# Autodesk Inventor assembly: Drive Roller Assembly 2
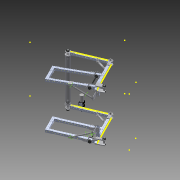
[picture p0: Inventor's stored thumbnail of the model, 180x180]
Saved by Autodesk Inventor 2014 (Build 180170000, 170)
## iProperties
Created: 2014-01-12
Part Number: Drive Roller Assembly 2
Document SubType Name: Assembly
Designer: Michael
Mass: 4835.9 g
Surface Area: 14934.6 cm^2
Volume: 1370.56 cm^3
Density: 3.52842 g/cm^3
Author: Michael
## Documents named in this file (33)
- C:\Users\Michael\Documents\GitHub\2014buildCAD\New Collector\Drive Roller Assembly 2.iam
- C:\Users\Michael\Documents\GitHub\2014buildCAD\Collector\Hex Shaft Collar 1-2 in (7552K500).ipt
- C:\Users\Michael\Documents\GitHub\2014buildCAD\Collector\Roller End Cap Drive (3-D Printed).ipt
- C:\Users\Michael\Documents\GitHub\2014buildCAD\Collector\Vex Pro VersaPlanetary Side Mount.ipt
- C:\Users\Michael\Documents\GitHub\2014buildCAD\Collector\VersaPlanetary (Fixed).iam
- C:\Users\Michael\Documents\GitHub\2014buildCAD\New Collector\Polycarbonate Roller 2 OD 1-16 Thick (8585K64).ipt
- C:\Users\Michael\Documents\GitHub\2014buildCAD\New Collector\Hex Bearing 1-2 in (FR8ZZ-Hex, am-0279).ipt
- C:\Users\Michael\Documents\GitHub\2014buildCAD\New Collector\Hex Shaft Collar 1-2 in (7552K500).ipt
- C:\Users\Michael\Documents\GitHub\2014buildCAD\New Collector\Roller End Cap Drive (3-D Printed).ipt
- C:\Users\Michael\Documents\GitHub\2014buildCAD\New Collector\Vex Pro End Bearing Mount.ipt
- C:\Users\Michael\Documents\GitHub\2014buildCAD\New Collector\Vex Pro 1x1 rectangular tubing 14 in length.ipt
- C:\Users\Michael\Documents\GitHub\2014buildCAD\New Collector\Hex Shaft Aluminum 1-2 in (am-2291).ipt
- C:\Users\Michael\Documents\GitHub\2014buildCAD\New Collector\Timing Pulley (HTD 5mm) - 18T 9mm Double Flange, 1-2 in Hex (VexPro).ipt
- C:\Users\Michael\Documents\GitHub\2014buildCAD\New Collector\Clamp with Piston Assembly.iam
- C:\Users\Michael\Documents\GitHub\2014buildCAD\New Collector\Vex Pro 90 degree gusset.ipt
- C:\Users\Michael\Documents\GitHub\2014buildCAD\New Collector\Vex Pro 1x1 rectangular tubing 2 in length.ipt
- C:\Users\Michael\Documents\GitHub\2014buildCAD\New Collector\Hex Shaft 3-8 in (am-0855).ipt
- C:\Users\Michael\Documents\GitHub\2014buildCAD\New Collector\Hex Shaft Collar 3-8 in (7552K300).ipt
- C:\Users\Michael\Documents\GitHub\2014buildCAD\New Collector\3 Postion Pneumatic Cylinder (9-16 in Bore, .25 in,2 in stroke).iam
- C:\Users\Michael\Documents\GitHub\2014buildCAD\New Collector\Hex Shaft 1-2 in (am-0856).ipt
- C:\Users\Michael\Documents\GitHub\2014buildCAD\New Collector\Spacer 2.ipt
- C:\Users\Michael\Documents\GitHub\2014buildCAD\New Collector\Gusset 3 (R-R) (Custom) ipt.ipt
- C:\Users\Michael\Documents\GitHub\2014buildCAD\New Collector\Gusset 3 (L-R) (Custom).ipt
- C:\Users\Michael\Documents\GitHub\2014buildCAD\New Collector\Gusset 3 (L-L) (Custom) ipt.ipt
- C:\Users\Michael\Documents\GitHub\2014buildCAD\New Collector\Gusset 3 (R-L) (Custom).ipt
- C:\Users\Michael\Documents\GitHub\2014buildCAD\New Collector\Vex Pro 1x1 rectangular tubing 4 in length.ipt
- C:\Users\Michael\Documents\GitHub\2014buildCAD\New Collector\Pneumatic Piston Back Flange (Lt Custom).ipt
- C:\Users\Michael\Documents\GitHub\2014buildCAD\New Collector\Pneumatic Piston Front Flange (Lt Custom).ipt
- C:\Users\Michael\Documents\GitHub\2014buildCAD\New Collector\Pneumatic Piston Front Flange (Rt Custom).ipt
- C:\Users\Michael\Documents\GitHub\2014buildCAD\New Collector\Pneumatic Piston Back Flange (Rt Custom).ipt
- C:\Users\Michael\Documents\GitHub\2014buildCAD\New Collector\Bearing Mount Spacer 1-8 in.ipt
- C:\Users\Michael\Documents\GitHub\2014buildCAD\New Collector\Vex Pro 1x1 rectangular tubing 14 in length (roller).ipt
- C:\Users\Michael\Documents\GitHub\2014buildCAD\New Collector\Complete Roller Pneumatic Cylinder Assembly.iam
## Components (95 placed, 30 different names)
1. Roller End Cap Drive (3-D Printed):2 — Mate:154, Mate:155, Mate:157, Mate:158, Mate:466, Mate:469
2. Vex Pro VersaPlanetary Side Mount:1 — Insert:29, Insert:30, Mate:564, Mate:565, Mate:566
3. VersaPlanetary (Fixed):1 [sub-assembly] — Insert:29, Insert:30, Mate:113, Mate:114, Mate:120, Mate:121, Mate:153
4. Hex Shaft Collar 1-2 in (7552K500):9 — Mate:113, Mate:114
5. Hex Shaft Collar 1-2 in (7552K500):10 — Mate:120, Mate:121
6. Polycarbonate Roller 2 OD 1-16 Thick (8585K64):3 — Mate:157, Mate:158, Mate:159, Mate:160
7. Hex Bearing 1-2 in (FR8ZZ-Hex, am-0279):3 — Mate:128, Mate:129, Mate:134, Mate:466
8. Roller End Cap Drive (3-D Printed):5 — Mate:159, Mate:160, Mate:632, Mate:635
9. Hex Shaft Aluminum 1-2 in (am-2291):1 — Flush:1, Mate:132, Mate:133, Mate:134, Mate:143, Mate:144, Mate:146, Mate:147, Mate:154, Mate:155, Mate:172, Mate:173, Mate:179, Mate:180, Mate:467, Mate:468
10. Vex Pro End Bearing Mount:4 — Mate:130, Mate:131, Mate:619, Mate:620, Mate:621
11. Vex Pro End Bearing Mount:5 — Mate:128, Mate:129, Mate:622, Mate:623, Mate:624
12. Hex Bearing 1-2 in (FR8ZZ-Hex, am-0279):4 — Mate:130, Mate:131, Flush:1, Mate:132, Mate:133, Mate:161
13. Timing Pulley (HTD 5mm) - 18T 9mm Double Flange, 1-2 in Hex (VexPro):3 — Mate:143, Mate:144, Mate:145, Mate:161
14. Hex Shaft Collar 1-2 in (7552K500):13 — Mate:145, Mate:146, Mate:147, Flush:2
15. Hex Shaft Collar 1-2 in (7552K500):14 — Flush:4, Mate:152
16. Timing Pulley (HTD 5mm) - 18T 9mm Double Flange, 1-2 in Hex (VexPro):4 — Mate:150, Flush:3, Mate:151, Flush:4, Mate:152
17. Hex Shaft Collar 1-2 in (7552K500):15 — Flush:2, Mate:150, Flush:3, Mate:151, Mate:153
18. Hex Bearing 1-2 in (FR8ZZ-Hex, am-0279):5 — Mate:178
19. Vex Pro End Bearing Mount:7 — Mate:626, Mate:630, Mate:631
20. Vex Pro End Bearing Mount:8 — Mate:627, Mate:628, Mate:629
21. Hex Bearing 1-2 in (FR8ZZ-Hex, am-0279):6 — Mate:172, Mate:173, Mate:470, Mate:471, Mate:632
22. Hex Shaft Collar 1-2 in (7552K500):16 — Mate:178, Mate:179, Mate:180, Flush:13
23. Clamp with Piston Assembly:1 [sub-assembly] — Mate:226, Mate:227, Flush:6, Mate:230, Mate:233, Mate:521, Mate:522, Mate:523
24. Vex Pro 1x1 rectangular tubing 14 in length:5 — Mate:203, Mate:210, Mate:211, Mate:221, Mate:222, Mate:223, Mate:264, Mate:265, Mate:266, Mate:267, Mate:268, Mate:269, Mate:326, Mate:328, Mate:329, Mate:427, Mate:429, Mate:611, Mate:612, Mate:615, Mate:616, Mate:617, Mate:618, Flush:20, Mate:644, Mate:648, Mate:649
25. Vex Pro 1x1 rectangular tubing 14 in length:6 — Mate:258, Mate:259, Mate:260, Mate:263, Mate:298, Mate:299, Mate:300, Mate:301, Mate:305, Mate:306, Mate:320, Mate:321, Mate:322, Mate:323, Mate:418, Mate:419, Mate:420, Mate:502, Mate:544, Mate:545, Mate:546, Mate:553, Mate:554, Mate:555, Flush:20, Mate:637, Mate:638, Mate:639, Mate:642
26. Vex Pro 90 degree gusset:8 — Mate:203, Mate:210, Mate:211, Mate:212, Mate:213, Mate:214
27. Vex Pro 1x1 rectangular tubing 2 in length:1 — Mate:212, Mate:213, Mate:214, Mate:327
28. Vex Pro 90 degree gusset:10 — Mate:221, Mate:222, Mate:223, Mate:433, Mate:434, Mate:435
29. Vex Pro 1x1 rectangular tubing 2 in length:2 — Mate:224, Mate:225, Flush:5, Mate:428
30. Hex Shaft 3-8 in (am-0855):1 — Mate:224, Mate:225, Flush:5, Mate:226, Mate:227, Flush:6, Mate:228, Mate:229, Mate:231, Mate:232
31. Hex Shaft Collar 3-8 in (7552K300):1 — Mate:228, Mate:229, Mate:230
32. Hex Shaft Collar 3-8 in (7552K300):2 — Mate:231, Mate:232, Mate:233
33. Clamp with Piston Assembly:2 [sub-assembly] — Mate:509, Mate:510, Mate:511
34. Vex Pro 90 degree gusset:11 — Mate:322, Mate:323, Mate:642
35. Vex Pro 90 degree gusset:12 — Mate:263, Mate:320, Mate:321, Mate:324, Mate:325
36. Vex Pro 1x1 rectangular tubing 2 in length:3 — Mate:324, Mate:325
37. Vex Pro 90 degree gusset:13 — Mate:258, Mate:259, Mate:260, Mate:425, Mate:426, Mate:492
38. Vex Pro 1x1 rectangular tubing 2 in length:4
39. Hex Shaft 3-8 in (am-0855):2
40. Hex Shaft Collar 3-8 in (7552K300):3
41. Hex Shaft Collar 3-8 in (7552K300):4
42. 3 Postion Pneumatic Cylinder (9-16 in Bore, .25 in,2 in stroke):1 [sub-assembly] — Mate:516, Mate:517, Mate:518, Mate:636
43. Vex Pro 90 degree gusset:14 — Mate:264, Mate:265, Mate:266, Mate:476, Mate:477, Mate:478
44. Vex Pro 90 degree gusset:15 — Mate:267, Mate:268, Mate:269
45. Vex Pro 90 degree gusset:17 — Mate:300, Mate:301, Mate:305, Mate:306, Mate:485, Mate:486, Mate:487
46. Vex Pro 90 degree gusset:18 — Mate:298, Mate:299, Mate:502
47. Vex Pro 90 degree gusset:19 — Mate:326, Mate:327, Mate:328, Mate:329
48. Hex Shaft 1-2 in (am-0856):2 — Mate:402, Mate:403, Mate:405, Mate:406, Mate:447, Mate:448, Flush:12
49. Hex Shaft Collar 1-2 in (7552K500):18 — Mate:402, Mate:403, Mate:450, Flush:12
50. Hex Shaft Collar 1-2 in (7552K500):19 — Mate:405, Mate:406, Mate:449
51. Hex Shaft 1-2 in (am-0856):3 — Mate:411, Mate:412, Flush:11, Mate:493, Mate:494, Mate:496, Mate:497
52. Hex Shaft Collar 1-2 in (7552K500):20 — Mate:411, Mate:412, Flush:11, Mate:495
53. Hex Shaft Collar 1-2 in (7552K500):21 — Mate:446, Mate:496, Mate:497
54. Spacer 2:1 — Mate:418, Mate:419, Mate:420, Mate:438, Mate:439, Mate:451, Mate:452, Mate:453
55. Gusset 3 (R-R) (Custom) ipt:1 — Mate:425, Mate:426, Mate:446, Mate:492
56. Spacer 2:2 — Mate:427, Mate:428, Mate:429, Mate:430, Mate:431, Mate:455, Mate:456, Mate:457
57. Gusset 3 (L-R) (Custom):1 — Mate:430, Mate:431, Mate:447, Mate:448, Mate:450, Mate:461
58. Gusset 3 (L-L) (Custom) ipt:1 — Mate:433, Mate:434, Mate:435, Mate:449
59. Gusset 3 (R-L) (Custom):1 — Mate:438, Mate:439, Mate:465, Mate:493, Mate:494, Mate:495
60. Spacer 2:3 — Mate:451, Mate:452, Mate:453, Mate:462, Mate:463, Mate:464
61. Spacer 2:4 — Mate:455, Mate:456, Mate:457, Mate:458, Mate:459, Mate:460
62. Spacer 2:5 — Mate:458, Mate:459, Mate:460, Mate:461
63. Spacer 2:6 — Mate:462, Mate:463, Mate:464, Mate:465
64. Hex Shaft Collar 1-2 in (7552K500):22 — Mate:467, Mate:468, Mate:469
65. Hex Shaft Aluminum 1-2 in (am-2291):2 — Mate:470, Mate:471, Flush:13, Mate:633, Mate:634
66. Vex Pro 1x1 rectangular tubing 4 in length:1 — Mate:476, Mate:477, Mate:478, Mate:513, Mate:514, Mate:515
67. Vex Pro 1x1 rectangular tubing 4 in length:2 — Mate:485, Mate:486, Mate:487, Mate:503, Mate:504, Mate:505
68. 3 Postion Pneumatic Cylinder (9-16 in Bore, .25 in,2 in stroke):2 [sub-assembly] — Mate:506, Mate:507, Mate:508, Mate:512
69. Pneumatic Piston Back Flange (Lt Custom):1 — Mate:503, Mate:504, Mate:505, Mate:506, Mate:507, Mate:508
70. Pneumatic Piston Front Flange (Lt Custom):1 — Mate:509, Mate:510, Mate:511, Mate:512
71. Pneumatic Piston Front Flange (Rt Custom):1 — Mate:521, Mate:522, Mate:523, Mate:636
72. Pneumatic Piston Back Flange (Rt Custom):1 — Mate:513, Mate:514, Mate:515, Mate:516, Mate:517, Mate:518
73. Vex Pro End Bearing Mount:9 — Mate:556, Mate:557
74. Bearing Mount Spacer 1-8 in:1
75. Bearing Mount Spacer 1-8 in:2 — Mate:544, Mate:545, Mate:546
76. Vex Pro End Bearing Mount:10 — Mate:558, Mate:559
77. Bearing Mount Spacer 1-8 in:3
78. Bearing Mount Spacer 1-8 in:4 — Mate:553, Mate:554, Mate:555
79. Hex Bearing 1-2 in (FR8ZZ-Hex, am-0279):7 — Mate:556, Mate:557, Flush:15, Mate:560, Mate:561, Mate:567
80. Hex Shaft 1-2 in (am-0856):4 — Mate:560, Mate:561, Mate:562, Mate:563
81. Hex Bearing 1-2 in (FR8ZZ-Hex, am-0279):8 — Mate:558, Mate:559, Flush:15
82. Vex Pro 1x1 rectangular tubing 14 in length (roller):1 — Mate:562, Mate:563, Mate:564, Mate:565, Mate:566, Mate:567, Mate:619, Mate:620, Mate:621, Mate:622, Mate:623, Mate:624, Flush:21, Mate:640, Mate:641
83. Vex Pro End Bearing Mount:11 — Mate:611, Mate:612
84. Bearing Mount Spacer 1-8 in:5
85. Bearing Mount Spacer 1-8 in:6 — Mate:618
86. Vex Pro End Bearing Mount:12
87. Bearing Mount Spacer 1-8 in:7
88. Bearing Mount Spacer 1-8 in:8 — Mate:615, Mate:616, Mate:617
89. Hex Bearing 1-2 in (FR8ZZ-Hex, am-0279):9 — Flush:19
90. Hex Shaft 1-2 in (am-0856):5 — Flush:19
91. Hex Bearing 1-2 in (FR8ZZ-Hex, am-0279):10
92. Vex Pro 1x1 rectangular tubing 14 in length (roller):2 — Mate:626, Mate:627, Mate:628, Mate:629, Mate:630, Mate:631, Flush:21, Mate:646, Mate:647
93. Hex Shaft Collar 1-2 in (7552K500):23 — Mate:633, Mate:634, Mate:635
94. Complete Roller Pneumatic Cylinder Assembly:1 [sub-assembly] — Mate:637, Mate:638, Mate:639, Mate:640, Mate:641
95. Complete Roller Pneumatic Cylinder Assembly:2 [sub-assembly] — Mate:644, Mate:646, Mate:647, Mate:648, Mate:649
## Relationships (281: Mate 263, Flush 16, Insert 2)
- Insert:29: Vex Pro VersaPlanetary Side Mount:1 ↔ VersaPlanetary (Fixed):1
- Insert:30: Vex Pro VersaPlanetary Side Mount:1 ↔ VersaPlanetary (Fixed):1
- Mate:113: VersaPlanetary (Fixed):1 ↔ Hex Shaft Collar 1-2 in (7552K500):9
- Mate:114: VersaPlanetary (Fixed):1 ↔ Hex Shaft Collar 1-2 in (7552K500):9
- Mate:120: VersaPlanetary (Fixed):1 ↔ Hex Shaft Collar 1-2 in (7552K500):10
- Mate:121: VersaPlanetary (Fixed):1 ↔ Hex Shaft Collar 1-2 in (7552K500):10
- Mate:128: Hex Bearing 1-2 in (FR8ZZ-Hex, am-0279):3 ↔ Vex Pro End Bearing Mount:5
- Mate:129: Hex Bearing 1-2 in (FR8ZZ-Hex, am-0279):3 ↔ Vex Pro End Bearing Mount:5
- Mate:130: Vex Pro End Bearing Mount:4 ↔ Hex Bearing 1-2 in (FR8ZZ-Hex, am-0279):4
- Mate:131: Vex Pro End Bearing Mount:4 ↔ Hex Bearing 1-2 in (FR8ZZ-Hex, am-0279):4
- Flush:1 (-25.4 mm): Hex Shaft Aluminum 1-2 in (am-2291):1 ↔ Hex Bearing 1-2 in (FR8ZZ-Hex, am-0279):4
- Mate:132: Hex Shaft Aluminum 1-2 in (am-2291):1 ↔ Hex Bearing 1-2 in (FR8ZZ-Hex, am-0279):4
- Mate:133: Hex Shaft Aluminum 1-2 in (am-2291):1 ↔ Hex Bearing 1-2 in (FR8ZZ-Hex, am-0279):4
- Mate:134: Hex Bearing 1-2 in (FR8ZZ-Hex, am-0279):3 ↔ Hex Shaft Aluminum 1-2 in (am-2291):1
- Mate:143: Hex Shaft Aluminum 1-2 in (am-2291):1 ↔ Timing Pulley (HTD 5mm) - 18T 9mm Double Flange, 1-2 in Hex (VexPro):3
- Mate:144: Hex Shaft Aluminum 1-2 in (am-2291):1 ↔ Timing Pulley (HTD 5mm) - 18T 9mm Double Flange, 1-2 in Hex (VexPro):3
- Mate:145: Timing Pulley (HTD 5mm) - 18T 9mm Double Flange, 1-2 in Hex (VexPro):3 ↔ Hex Shaft Collar 1-2 in (7552K500):13
- Mate:146: Hex Shaft Aluminum 1-2 in (am-2291):1 ↔ Hex Shaft Collar 1-2 in (7552K500):13
- Mate:147: Hex Shaft Aluminum 1-2 in (am-2291):1 ↔ Hex Shaft Collar 1-2 in (7552K500):13
- [Mate]: Hex Shaft Collar 1-2 in (7552K500):14 ↔ Timing Pulley (HTD 5mm) - 18T 9mm Double Flange, 1-2 in Hex (VexPro):4
- [Mate]: Timing Pulley (HTD 5mm) - 18T 9mm Double Flange, 1-2 in Hex (VexPro):4 ↔ Hex Shaft Collar 1-2 in (7552K500):15
- Flush:2: Hex Shaft Collar 1-2 in (7552K500):13 ↔ Hex Shaft Collar 1-2 in (7552K500):15
- Mate:150: Timing Pulley (HTD 5mm) - 18T 9mm Double Flange, 1-2 in Hex (VexPro):4 ↔ Hex Shaft Collar 1-2 in (7552K500):15
- Flush:3: Timing Pulley (HTD 5mm) - 18T 9mm Double Flange, 1-2 in Hex (VexPro):4 ↔ Hex Shaft Collar 1-2 in (7552K500):15
- Mate:151: Timing Pulley (HTD 5mm) - 18T 9mm Double Flange, 1-2 in Hex (VexPro):4 ↔ Hex Shaft Collar 1-2 in (7552K500):15
- Flush:4: Hex Shaft Collar 1-2 in (7552K500):14 ↔ Timing Pulley (HTD 5mm) - 18T 9mm Double Flange, 1-2 in Hex (VexPro):4
- Mate:152: Hex Shaft Collar 1-2 in (7552K500):14 ↔ Timing Pulley (HTD 5mm) - 18T 9mm Double Flange, 1-2 in Hex (VexPro):4
- Mate:153: VersaPlanetary (Fixed):1 ↔ Hex Shaft Collar 1-2 in (7552K500):15
- Mate:154: Roller End Cap Drive (3-D Printed):2 ↔ Hex Shaft Aluminum 1-2 in (am-2291):1
- Mate:155: Roller End Cap Drive (3-D Printed):2 ↔ Hex Shaft Aluminum 1-2 in (am-2291):1
- Mate:157: Roller End Cap Drive (3-D Printed):2 ↔ Polycarbonate Roller 2 OD 1-16 Thick (8585K64):3
- Mate:158: Roller End Cap Drive (3-D Printed):2 ↔ Polycarbonate Roller 2 OD 1-16 Thick (8585K64):3
- Mate:159: Polycarbonate Roller 2 OD 1-16 Thick (8585K64):3 ↔ Roller End Cap Drive (3-D Printed):5
- Mate:160: Polycarbonate Roller 2 OD 1-16 Thick (8585K64):3 ↔ Roller End Cap Drive (3-D Printed):5
- Mate:161: Hex Bearing 1-2 in (FR8ZZ-Hex, am-0279):4 ↔ Timing Pulley (HTD 5mm) - 18T 9mm Double Flange, 1-2 in Hex (VexPro):3
- [Mate]: Hex Bearing 1-2 in (FR8ZZ-Hex, am-0279):5 ↔ Vex Pro End Bearing Mount:8
- [Mate]: Hex Bearing 1-2 in (FR8ZZ-Hex, am-0279):5 ↔ Vex Pro End Bearing Mount:8
- [Mate]: Vex Pro End Bearing Mount:7 ↔ Hex Bearing 1-2 in (FR8ZZ-Hex, am-0279):6
- [Mate]: Vex Pro End Bearing Mount:7 ↔ Hex Bearing 1-2 in (FR8ZZ-Hex, am-0279):6
- Mate:172: Hex Shaft Aluminum 1-2 in (am-2291):1 ↔ Hex Bearing 1-2 in (FR8ZZ-Hex, am-0279):6
- Mate:173: Hex Shaft Aluminum 1-2 in (am-2291):1 ↔ Hex Bearing 1-2 in (FR8ZZ-Hex, am-0279):6
- Mate:178: Hex Bearing 1-2 in (FR8ZZ-Hex, am-0279):5 ↔ Hex Shaft Collar 1-2 in (7552K500):16
- Mate:179: Hex Shaft Aluminum 1-2 in (am-2291):1 ↔ Hex Shaft Collar 1-2 in (7552K500):16
- Mate:180: Hex Shaft Aluminum 1-2 in (am-2291):1 ↔ Hex Shaft Collar 1-2 in (7552K500):16
- Mate:203: Vex Pro 1x1 rectangular tubing 14 in length:5 ↔ Vex Pro 90 degree gusset:8
- Mate:210: Vex Pro 1x1 rectangular tubing 14 in length:5 ↔ Vex Pro 90 degree gusset:8
- Mate:211: Vex Pro 1x1 rectangular tubing 14 in length:5 ↔ Vex Pro 90 degree gusset:8
- Mate:212: Vex Pro 90 degree gusset:8 ↔ Vex Pro 1x1 rectangular tubing 2 in length:1
- Mate:213: Vex Pro 90 degree gusset:8 ↔ Vex Pro 1x1 rectangular tubing 2 in length:1
- Mate:214: Vex Pro 90 degree gusset:8 ↔ Vex Pro 1x1 rectangular tubing 2 in length:1
- [Mate]: Vex Pro 90 degree gusset:10 ↔ Vex Pro 1x1 rectangular tubing 2 in length:2
- [Mate]: Vex Pro 90 degree gusset:10 ↔ Vex Pro 1x1 rectangular tubing 2 in length:2
- [Mate]: Vex Pro 90 degree gusset:10 ↔ Vex Pro 1x1 rectangular tubing 2 in length:2
- Mate:221: Vex Pro 1x1 rectangular tubing 14 in length:5 ↔ Vex Pro 90 degree gusset:10
- Mate:222: Vex Pro 1x1 rectangular tubing 14 in length:5 ↔ Vex Pro 90 degree gusset:10
- Mate:223: Vex Pro 1x1 rectangular tubing 14 in length:5 ↔ Vex Pro 90 degree gusset:10
- Mate:224: Vex Pro 1x1 rectangular tubing 2 in length:2 ↔ Hex Shaft 3-8 in (am-0855):1
- Mate:225: Vex Pro 1x1 rectangular tubing 2 in length:2 ↔ Hex Shaft 3-8 in (am-0855):1
- Flush:5 (-19.05 mm): Vex Pro 1x1 rectangular tubing 2 in length:2 ↔ Hex Shaft 3-8 in (am-0855):1
- Mate:226: Clamp with Piston Assembly:1 ↔ Hex Shaft 3-8 in (am-0855):1
- Mate:227: Clamp with Piston Assembly:1 ↔ Hex Shaft 3-8 in (am-0855):1
- Flush:6 (-9.525 mm): Clamp with Piston Assembly:1 ↔ Hex Shaft 3-8 in (am-0855):1
- Mate:228: Hex Shaft 3-8 in (am-0855):1 ↔ Hex Shaft Collar 3-8 in (7552K300):1
- Mate:229: Hex Shaft 3-8 in (am-0855):1 ↔ Hex Shaft Collar 3-8 in (7552K300):1
- Mate:230: Clamp with Piston Assembly:1 ↔ Hex Shaft Collar 3-8 in (7552K300):1
- Mate:231: Hex Shaft 3-8 in (am-0855):1 ↔ Hex Shaft Collar 3-8 in (7552K300):2
- Mate:232: Hex Shaft 3-8 in (am-0855):1 ↔ Hex Shaft Collar 3-8 in (7552K300):2
- Mate:233: Clamp with Piston Assembly:1 ↔ Hex Shaft Collar 3-8 in (7552K300):2
- [Mate]: Vex Pro 90 degree gusset:12 ↔ Vex Pro 1x1 rectangular tubing 2 in length:3
- [Mate]: Vex Pro 90 degree gusset:13 ↔ Vex Pro 1x1 rectangular tubing 2 in length:4
- [Mate]: Vex Pro 90 degree gusset:13 ↔ Vex Pro 1x1 rectangular tubing 2 in length:4
- [Mate]: Vex Pro 90 degree gusset:13 ↔ Vex Pro 1x1 rectangular tubing 2 in length:4
- [Mate]: Vex Pro 1x1 rectangular tubing 2 in length:4 ↔ Hex Shaft 3-8 in (am-0855):2
- [Mate]: Vex Pro 1x1 rectangular tubing 2 in length:4 ↔ Hex Shaft 3-8 in (am-0855):2
- [Flush] (-19.05 mm): Vex Pro 1x1 rectangular tubing 2 in length:4 ↔ Hex Shaft 3-8 in (am-0855):2
- [Mate]: Clamp with Piston Assembly:2 ↔ Hex Shaft 3-8 in (am-0855):2
- [Mate]: Clamp with Piston Assembly:2 ↔ Hex Shaft 3-8 in (am-0855):2
- [Flush] (-9.525 mm): Clamp with Piston Assembly:2 ↔ Hex Shaft 3-8 in (am-0855):2
- [Mate]: Hex Shaft 3-8 in (am-0855):2 ↔ Hex Shaft Collar 3-8 in (7552K300):3
- [Mate]: Hex Shaft 3-8 in (am-0855):2 ↔ Hex Shaft Collar 3-8 in (7552K300):3
- [Mate]: Clamp with Piston Assembly:2 ↔ Hex Shaft Collar 3-8 in (7552K300):3
- [Mate]: Hex Shaft 3-8 in (am-0855):2 ↔ Hex Shaft Collar 3-8 in (7552K300):4
- [Mate]: Hex Shaft 3-8 in (am-0855):2 ↔ Hex Shaft Collar 3-8 in (7552K300):4
- [Mate]: Clamp with Piston Assembly:2 ↔ Hex Shaft Collar 3-8 in (7552K300):4
- Mate:258: Vex Pro 1x1 rectangular tubing 14 in length:6 ↔ Vex Pro 90 degree gusset:13
- Mate:259: Vex Pro 1x1 rectangular tubing 14 in length:6 ↔ Vex Pro 90 degree gusset:13
- Mate:260: Vex Pro 1x1 rectangular tubing 14 in length:6 ↔ Vex Pro 90 degree gusset:13
- Mate:263: Vex Pro 1x1 rectangular tubing 14 in length:6 ↔ Vex Pro 90 degree gusset:12
- Mate:264: Vex Pro 1x1 rectangular tubing 14 in length:5 ↔ Vex Pro 90 degree gusset:14
- Mate:265: Vex Pro 1x1 rectangular tubing 14 in length:5 ↔ Vex Pro 90 degree gusset:14
- Mate:266: Vex Pro 1x1 rectangular tubing 14 in length:5 ↔ Vex Pro 90 degree gusset:14
- Mate:267: Vex Pro 1x1 rectangular tubing 14 in length:5 ↔ Vex Pro 90 degree gusset:15
- Mate:268: Vex Pro 1x1 rectangular tubing 14 in length:5 ↔ Vex Pro 90 degree gusset:15
- Mate:269: Vex Pro 1x1 rectangular tubing 14 in length:5 ↔ Vex Pro 90 degree gusset:15
- Mate:298: Vex Pro 1x1 rectangular tubing 14 in length:6 ↔ Vex Pro 90 degree gusset:18
- Mate:299: Vex Pro 1x1 rectangular tubing 14 in length:6 ↔ Vex Pro 90 degree gusset:18
- Mate:300: Vex Pro 1x1 rectangular tubing 14 in length:6 ↔ Vex Pro 90 degree gusset:17
- Mate:301: Vex Pro 1x1 rectangular tubing 14 in length:6 ↔ Vex Pro 90 degree gusset:17
- Mate:305: Vex Pro 1x1 rectangular tubing 14 in length:6 ↔ Vex Pro 90 degree gusset:17
- Mate:306: Vex Pro 1x1 rectangular tubing 14 in length:6 ↔ Vex Pro 90 degree gusset:17
- Mate:320: Vex Pro 1x1 rectangular tubing 14 in length:6 ↔ Vex Pro 90 degree gusset:12
- Mate:321: Vex Pro 1x1 rectangular tubing 14 in length:6 ↔ Vex Pro 90 degree gusset:12
- Mate:322: Vex Pro 1x1 rectangular tubing 14 in length:6 ↔ Vex Pro 90 degree gusset:11
- Mate:323: Vex Pro 1x1 rectangular tubing 14 in length:6 ↔ Vex Pro 90 degree gusset:11
- Mate:324: Vex Pro 90 degree gusset:12 ↔ Vex Pro 1x1 rectangular tubing 2 in length:3
- Mate:325: Vex Pro 90 degree gusset:12 ↔ Vex Pro 1x1 rectangular tubing 2 in length:3
- Mate:326: Vex Pro 1x1 rectangular tubing 14 in length:5 ↔ Vex Pro 90 degree gusset:19
- Mate:327: Vex Pro 1x1 rectangular tubing 2 in length:1 ↔ Vex Pro 90 degree gusset:19
- Mate:328: Vex Pro 1x1 rectangular tubing 14 in length:5 ↔ Vex Pro 90 degree gusset:19
- Mate:329: Vex Pro 1x1 rectangular tubing 14 in length:5 ↔ Vex Pro 90 degree gusset:19
- Mate:402: Hex Shaft 1-2 in (am-0856):2 ↔ Hex Shaft Collar 1-2 in (7552K500):18
- Mate:403: Hex Shaft 1-2 in (am-0856):2 ↔ Hex Shaft Collar 1-2 in (7552K500):18
- Mate:405: Hex Shaft 1-2 in (am-0856):2 ↔ Hex Shaft Collar 1-2 in (7552K500):19
- Mate:406: Hex Shaft 1-2 in (am-0856):2 ↔ Hex Shaft Collar 1-2 in (7552K500):19
- Mate:411: Hex Shaft 1-2 in (am-0856):3 ↔ Hex Shaft Collar 1-2 in (7552K500):20
- Mate:412: Hex Shaft 1-2 in (am-0856):3 ↔ Hex Shaft Collar 1-2 in (7552K500):20
- Flush:11 (-9.525 mm): Hex Shaft 1-2 in (am-0856):3 ↔ Hex Shaft Collar 1-2 in (7552K500):20
- Mate:418: Vex Pro 1x1 rectangular tubing 14 in length:6 ↔ Spacer 2:1
- Mate:419: Vex Pro 1x1 rectangular tubing 14 in length:6 ↔ Spacer 2:1
- Mate:420: Vex Pro 1x1 rectangular tubing 14 in length:6 ↔ Spacer 2:1
- Mate:425: Vex Pro 90 degree gusset:13 ↔ Gusset 3 (R-R) (Custom) ipt:1
- Mate:426: Vex Pro 90 degree gusset:13 ↔ Gusset 3 (R-R) (Custom) ipt:1
- Mate:427: Vex Pro 1x1 rectangular tubing 14 in length:5 ↔ Spacer 2:2
- Mate:428: Vex Pro 1x1 rectangular tubing 2 in length:2 ↔ Spacer 2:2
- Mate:429: Vex Pro 1x1 rectangular tubing 14 in length:5 ↔ Spacer 2:2
- Mate:430: Spacer 2:2 ↔ Gusset 3 (L-R) (Custom):1
- Mate:431: Spacer 2:2 ↔ Gusset 3 (L-R) (Custom):1
- Mate:433: Vex Pro 90 degree gusset:10 ↔ Gusset 3 (L-L) (Custom) ipt:1
- Mate:434: Vex Pro 90 degree gusset:10 ↔ Gusset 3 (L-L) (Custom) ipt:1
- Mate:435: Vex Pro 90 degree gusset:10 ↔ Gusset 3 (L-L) (Custom) ipt:1
- Mate:438: Spacer 2:1 ↔ Gusset 3 (R-L) (Custom):1
- Mate:439: Spacer 2:1 ↔ Gusset 3 (R-L) (Custom):1
- Mate:446: Hex Shaft Collar 1-2 in (7552K500):21 ↔ Gusset 3 (R-R) (Custom) ipt:1
- Mate:447: Hex Shaft 1-2 in (am-0856):2 ↔ Gusset 3 (L-R) (Custom):1
- Mate:448: Hex Shaft 1-2 in (am-0856):2 ↔ Gusset 3 (L-R) (Custom):1
- Mate:449: Hex Shaft Collar 1-2 in (7552K500):19 ↔ Gusset 3 (L-L) (Custom) ipt:1
- Mate:450: Hex Shaft Collar 1-2 in (7552K500):18 ↔ Gusset 3 (L-R) (Custom):1
- Mate:451: Spacer 2:1 ↔ Spacer 2:3
- Mate:452: Spacer 2:1 ↔ Spacer 2:3
- Mate:453: Spacer 2:1 ↔ Spacer 2:3
- Mate:455: Spacer 2:2 ↔ Spacer 2:4
- Mate:456: Spacer 2:2 ↔ Spacer 2:4
- Mate:457: Spacer 2:2 ↔ Spacer 2:4
- Mate:458: Spacer 2:4 ↔ Spacer 2:5
- Mate:459: Spacer 2:4 ↔ Spacer 2:5
- Mate:460: Spacer 2:4 ↔ Spacer 2:5
- Mate:461: Gusset 3 (L-R) (Custom):1 ↔ Spacer 2:5
- Mate:462: Spacer 2:3 ↔ Spacer 2:6
- Mate:463: Spacer 2:3 ↔ Spacer 2:6
- Mate:464: Spacer 2:3 ↔ Spacer 2:6
- Mate:465: Gusset 3 (R-L) (Custom):1 ↔ Spacer 2:6
- Flush:12 (-9.525 mm): Hex Shaft 1-2 in (am-0856):2 ↔ Hex Shaft Collar 1-2 in (7552K500):18
- Mate:466: Roller End Cap Drive (3-D Printed):2 ↔ Hex Bearing 1-2 in (FR8ZZ-Hex, am-0279):3
- Mate:467: Hex Shaft Aluminum 1-2 in (am-2291):1 ↔ Hex Shaft Collar 1-2 in (7552K500):22
- Mate:468: Hex Shaft Aluminum 1-2 in (am-2291):1 ↔ Hex Shaft Collar 1-2 in (7552K500):22
- Mate:469: Roller End Cap Drive (3-D Printed):2 ↔ Hex Shaft Collar 1-2 in (7552K500):22
- Mate:470: Hex Bearing 1-2 in (FR8ZZ-Hex, am-0279):6 ↔ Hex Shaft Aluminum 1-2 in (am-2291):2
- Mate:471: Hex Bearing 1-2 in (FR8ZZ-Hex, am-0279):6 ↔ Hex Shaft Aluminum 1-2 in (am-2291):2
- Flush:13 (-3.175 mm): Hex Shaft Collar 1-2 in (7552K500):16 ↔ Hex Shaft Aluminum 1-2 in (am-2291):2
- Mate:476: Vex Pro 90 degree gusset:14 ↔ Vex Pro 1x1 rectangular tubing 4 in length:1
- Mate:477: Vex Pro 90 degree gusset:14 ↔ Vex Pro 1x1 rectangular tubing 4 in length:1
- Mate:478: Vex Pro 90 degree gusset:14 ↔ Vex Pro 1x1 rectangular tubing 4 in length:1
- Mate:485: Vex Pro 90 degree gusset:17 ↔ Vex Pro 1x1 rectangular tubing 4 in length:2
- Mate:486: Vex Pro 90 degree gusset:17 ↔ Vex Pro 1x1 rectangular tubing 4 in length:2
- Mate:487: Vex Pro 90 degree gusset:17 ↔ Vex Pro 1x1 rectangular tubing 4 in length:2
- Mate:492: Vex Pro 90 degree gusset:13 ↔ Gusset 3 (R-R) (Custom) ipt:1
- Mate:493: Hex Shaft 1-2 in (am-0856):3 ↔ Gusset 3 (R-L) (Custom):1
- Mate:494: Hex Shaft 1-2 in (am-0856):3 ↔ Gusset 3 (R-L) (Custom):1
- Mate:495: Hex Shaft Collar 1-2 in (7552K500):20 ↔ Gusset 3 (R-L) (Custom):1
- Mate:496: Hex Shaft 1-2 in (am-0856):3 ↔ Hex Shaft Collar 1-2 in (7552K500):21
- Mate:497: Hex Shaft 1-2 in (am-0856):3 ↔ Hex Shaft Collar 1-2 in (7552K500):21
- Mate:502: Vex Pro 1x1 rectangular tubing 14 in length:6 ↔ Vex Pro 90 degree gusset:18
- Mate:503: Vex Pro 1x1 rectangular tubing 4 in length:2 ↔ Pneumatic Piston Back Flange (Lt Custom):1
- Mate:504: Vex Pro 1x1 rectangular tubing 4 in length:2 ↔ Pneumatic Piston Back Flange (Lt Custom):1
- Mate:505: Vex Pro 1x1 rectangular tubing 4 in length:2 ↔ Pneumatic Piston Back Flange (Lt Custom):1
- Mate:506: 3 Postion Pneumatic Cylinder (9-16 in Bore, .25 in,2 in stroke):2 ↔ Pneumatic Piston Back Flange (Lt Custom):1
- Mate:507: 3 Postion Pneumatic Cylinder (9-16 in Bore, .25 in,2 in stroke):2 ↔ Pneumatic Piston Back Flange (Lt Custom):1
- Mate:508: 3 Postion Pneumatic Cylinder (9-16 in Bore, .25 in,2 in stroke):2 ↔ Pneumatic Piston Back Flange (Lt Custom):1
- Mate:509: Clamp with Piston Assembly:2 ↔ Pneumatic Piston Front Flange (Lt Custom):1
- Mate:510: Clamp with Piston Assembly:2 ↔ Pneumatic Piston Front Flange (Lt Custom):1
- Mate:511: Clamp with Piston Assembly:2 ↔ Pneumatic Piston Front Flange (Lt Custom):1
- Mate:512: 3 Postion Pneumatic Cylinder (9-16 in Bore, .25 in,2 in stroke):2 ↔ Pneumatic Piston Front Flange (Lt Custom):1
- Mate:513: Vex Pro 1x1 rectangular tubing 4 in length:1 ↔ Pneumatic Piston Back Flange (Rt Custom):1
- Mate:514: Vex Pro 1x1 rectangular tubing 4 in length:1 ↔ Pneumatic Piston Back Flange (Rt Custom):1
- Mate:515: Vex Pro 1x1 rectangular tubing 4 in length:1 ↔ Pneumatic Piston Back Flange (Rt Custom):1
- Mate:516: 3 Postion Pneumatic Cylinder (9-16 in Bore, .25 in,2 in stroke):1 ↔ Pneumatic Piston Back Flange (Rt Custom):1
- Mate:517: 3 Postion Pneumatic Cylinder (9-16 in Bore, .25 in,2 in stroke):1 ↔ Pneumatic Piston Back Flange (Rt Custom):1
- Mate:518: 3 Postion Pneumatic Cylinder (9-16 in Bore, .25 in,2 in stroke):1 ↔ Pneumatic Piston Back Flange (Rt Custom):1
- Mate:521: Clamp with Piston Assembly:1 ↔ Pneumatic Piston Front Flange (Rt Custom):1
- Mate:522: Clamp with Piston Assembly:1 ↔ Pneumatic Piston Front Flange (Rt Custom):1
- Mate:523: Clamp with Piston Assembly:1 ↔ Pneumatic Piston Front Flange (Rt Custom):1
- [Mate]: Vex Pro End Bearing Mount:9 ↔ Bearing Mount Spacer 1-8 in:1
- [Mate]: Vex Pro End Bearing Mount:9 ↔ Bearing Mount Spacer 1-8 in:1
- [Mate]: Vex Pro End Bearing Mount:9 ↔ Bearing Mount Spacer 1-8 in:1
- [Mate]: Bearing Mount Spacer 1-8 in:1 ↔ Bearing Mount Spacer 1-8 in:2
- [Mate]: Bearing Mount Spacer 1-8 in:1 ↔ Bearing Mount Spacer 1-8 in:2
- [Mate]: Bearing Mount Spacer 1-8 in:1 ↔ Bearing Mount Spacer 1-8 in:2
- Mate:544: Vex Pro 1x1 rectangular tubing 14 in length:6 ↔ Bearing Mount Spacer 1-8 in:2
- Mate:545: Vex Pro 1x1 rectangular tubing 14 in length:6 ↔ Bearing Mount Spacer 1-8 in:2
- Mate:546: Vex Pro 1x1 rectangular tubing 14 in length:6 ↔ Bearing Mount Spacer 1-8 in:2
- [Mate]: Vex Pro End Bearing Mount:10 ↔ Bearing Mount Spacer 1-8 in:3
- [Mate]: Vex Pro End Bearing Mount:10 ↔ Bearing Mount Spacer 1-8 in:3
- [Mate]: Vex Pro End Bearing Mount:10 ↔ Bearing Mount Spacer 1-8 in:3
- [Mate]: Bearing Mount Spacer 1-8 in:3 ↔ Bearing Mount Spacer 1-8 in:4
- [Mate]: Bearing Mount Spacer 1-8 in:3 ↔ Bearing Mount Spacer 1-8 in:4
- [Mate]: Bearing Mount Spacer 1-8 in:3 ↔ Bearing Mount Spacer 1-8 in:4
- Mate:553: Vex Pro 1x1 rectangular tubing 14 in length:6 ↔ Bearing Mount Spacer 1-8 in:4
- Mate:554: Vex Pro 1x1 rectangular tubing 14 in length:6 ↔ Bearing Mount Spacer 1-8 in:4
- Mate:555: Vex Pro 1x1 rectangular tubing 14 in length:6 ↔ Bearing Mount Spacer 1-8 in:4
- Mate:556: Vex Pro End Bearing Mount:9 ↔ Hex Bearing 1-2 in (FR8ZZ-Hex, am-0279):7
- Mate:557: Vex Pro End Bearing Mount:9 ↔ Hex Bearing 1-2 in (FR8ZZ-Hex, am-0279):7
- Mate:558: Vex Pro End Bearing Mount:10 ↔ Hex Bearing 1-2 in (FR8ZZ-Hex, am-0279):8
- Mate:559: Vex Pro End Bearing Mount:10 ↔ Hex Bearing 1-2 in (FR8ZZ-Hex, am-0279):8
- Flush:15: Hex Bearing 1-2 in (FR8ZZ-Hex, am-0279):7 ↔ Hex Bearing 1-2 in (FR8ZZ-Hex, am-0279):8
- Mate:560: Hex Bearing 1-2 in (FR8ZZ-Hex, am-0279):7 ↔ Hex Shaft 1-2 in (am-0856):4
- Mate:561: Hex Bearing 1-2 in (FR8ZZ-Hex, am-0279):7 ↔ Hex Shaft 1-2 in (am-0856):4
- Mate:562: Hex Shaft 1-2 in (am-0856):4 ↔ Vex Pro 1x1 rectangular tubing 14 in length (roller):1
- Mate:563: Hex Shaft 1-2 in (am-0856):4 ↔ Vex Pro 1x1 rectangular tubing 14 in length (roller):1
- Mate:564: Vex Pro VersaPlanetary Side Mount:1 ↔ Vex Pro 1x1 rectangular tubing 14 in length (roller):1
- Mate:565: Vex Pro VersaPlanetary Side Mount:1 ↔ Vex Pro 1x1 rectangular tubing 14 in length (roller):1
- Mate:566: Vex Pro VersaPlanetary Side Mount:1 ↔ Vex Pro 1x1 rectangular tubing 14 in length (roller):1
- Mate:567 (2.3813 mm): Hex Bearing 1-2 in (FR8ZZ-Hex, am-0279):7 ↔ Vex Pro 1x1 rectangular tubing 14 in length (roller):1
- [Mate]: Vex Pro End Bearing Mount:11 ↔ Bearing Mount Spacer 1-8 in:5
- [Mate]: Vex Pro End Bearing Mount:11 ↔ Bearing Mount Spacer 1-8 in:5
- [Mate]: Vex Pro End Bearing Mount:11 ↔ Bearing Mount Spacer 1-8 in:5
- [Mate]: Bearing Mount Spacer 1-8 in:5 ↔ Bearing Mount Spacer 1-8 in:6
- [Mate]: Bearing Mount Spacer 1-8 in:5 ↔ Bearing Mount Spacer 1-8 in:6
- [Mate]: Bearing Mount Spacer 1-8 in:5 ↔ Bearing Mount Spacer 1-8 in:6
- [Mate]: Vex Pro End Bearing Mount:12 ↔ Bearing Mount Spacer 1-8 in:7
- [Mate]: Vex Pro End Bearing Mount:12 ↔ Bearing Mount Spacer 1-8 in:7
- [Mate]: Vex Pro End Bearing Mount:12 ↔ Bearing Mount Spacer 1-8 in:7
- [Mate]: Bearing Mount Spacer 1-8 in:7 ↔ Bearing Mount Spacer 1-8 in:8
- [Mate]: Bearing Mount Spacer 1-8 in:7 ↔ Bearing Mount Spacer 1-8 in:8
- [Mate]: Bearing Mount Spacer 1-8 in:7 ↔ Bearing Mount Spacer 1-8 in:8
- [Mate]: Vex Pro End Bearing Mount:11 ↔ Hex Bearing 1-2 in (FR8ZZ-Hex, am-0279):9
- [Mate]: Vex Pro End Bearing Mount:11 ↔ Hex Bearing 1-2 in (FR8ZZ-Hex, am-0279):9
- [Mate]: Vex Pro End Bearing Mount:12 ↔ Hex Bearing 1-2 in (FR8ZZ-Hex, am-0279):10
- [Mate]: Vex Pro End Bearing Mount:12 ↔ Hex Bearing 1-2 in (FR8ZZ-Hex, am-0279):10
- [Flush]: Hex Bearing 1-2 in (FR8ZZ-Hex, am-0279):9 ↔ Hex Bearing 1-2 in (FR8ZZ-Hex, am-0279):10
- [Mate]: Hex Bearing 1-2 in (FR8ZZ-Hex, am-0279):9 ↔ Hex Shaft 1-2 in (am-0856):5
- [Mate]: Hex Bearing 1-2 in (FR8ZZ-Hex, am-0279):9 ↔ Hex Shaft 1-2 in (am-0856):5
- [Mate]: Hex Shaft 1-2 in (am-0856):5 ↔ Vex Pro 1x1 rectangular tubing 14 in length (roller):2
- [Mate]: Hex Shaft 1-2 in (am-0856):5 ↔ Vex Pro 1x1 rectangular tubing 14 in length (roller):2
- [Mate] (2.3813 mm): Hex Bearing 1-2 in (FR8ZZ-Hex, am-0279):9 ↔ Vex Pro 1x1 rectangular tubing 14 in length (roller):2
- Mate:611: Vex Pro 1x1 rectangular tubing 14 in length:5 ↔ Vex Pro End Bearing Mount:11
- Mate:612: Vex Pro 1x1 rectangular tubing 14 in length:5 ↔ Vex Pro End Bearing Mount:11
- Mate:615: Vex Pro 1x1 rectangular tubing 14 in length:5 ↔ Bearing Mount Spacer 1-8 in:8
- Mate:616: Vex Pro 1x1 rectangular tubing 14 in length:5 ↔ Bearing Mount Spacer 1-8 in:8
- Mate:617: Vex Pro 1x1 rectangular tubing 14 in length:5 ↔ Bearing Mount Spacer 1-8 in:8
- Mate:618: Vex Pro 1x1 rectangular tubing 14 in length:5 ↔ Bearing Mount Spacer 1-8 in:6
- Flush:19 (15.0812 mm): Hex Bearing 1-2 in (FR8ZZ-Hex, am-0279):9 ↔ Hex Shaft 1-2 in (am-0856):5
- Mate:619: Vex Pro End Bearing Mount:4 ↔ Vex Pro 1x1 rectangular tubing 14 in length (roller):1
- Mate:620: Vex Pro End Bearing Mount:4 ↔ Vex Pro 1x1 rectangular tubing 14 in length (roller):1
- Mate:621: Vex Pro End Bearing Mount:4 ↔ Vex Pro 1x1 rectangular tubing 14 in length (roller):1
- Mate:622: Vex Pro End Bearing Mount:5 ↔ Vex Pro 1x1 rectangular tubing 14 in length (roller):1
- Mate:623: Vex Pro End Bearing Mount:5 ↔ Vex Pro 1x1 rectangular tubing 14 in length (roller):1
- Mate:624: Vex Pro End Bearing Mount:5 ↔ Vex Pro 1x1 rectangular tubing 14 in length (roller):1
- Mate:626: Vex Pro End Bearing Mount:7 ↔ Vex Pro 1x1 rectangular tubing 14 in length (roller):2
- Mate:627: Vex Pro End Bearing Mount:8 ↔ Vex Pro 1x1 rectangular tubing 14 in length (roller):2
- Mate:628: Vex Pro End Bearing Mount:8 ↔ Vex Pro 1x1 rectangular tubing 14 in length (roller):2
- Mate:629: Vex Pro End Bearing Mount:8 ↔ Vex Pro 1x1 rectangular tubing 14 in length (roller):2
- Flush:20: Vex Pro 1x1 rectangular tubing 14 in length:5 ↔ Vex Pro 1x1 rectangular tubing 14 in length:6
- Mate:630: Vex Pro End Bearing Mount:7 ↔ Vex Pro 1x1 rectangular tubing 14 in length (roller):2
- Mate:631: Vex Pro End Bearing Mount:7 ↔ Vex Pro 1x1 rectangular tubing 14 in length (roller):2
- Mate:632: Roller End Cap Drive (3-D Printed):5 ↔ Hex Bearing 1-2 in (FR8ZZ-Hex, am-0279):6
- Mate:633: Hex Shaft Aluminum 1-2 in (am-2291):2 ↔ Hex Shaft Collar 1-2 in (7552K500):23
- Mate:634: Hex Shaft Aluminum 1-2 in (am-2291):2 ↔ Hex Shaft Collar 1-2 in (7552K500):23
- Mate:635: Roller End Cap Drive (3-D Printed):5 ↔ Hex Shaft Collar 1-2 in (7552K500):23
- Flush:21: Vex Pro 1x1 rectangular tubing 14 in length (roller):1 ↔ Vex Pro 1x1 rectangular tubing 14 in length (roller):2
- Mate:636: 3 Postion Pneumatic Cylinder (9-16 in Bore, .25 in,2 in stroke):1 ↔ Pneumatic Piston Front Flange (Rt Custom):1
- Mate:637: Vex Pro 1x1 rectangular tubing 14 in length:6 ↔ Complete Roller Pneumatic Cylinder Assembly:1
- Mate:638: Vex Pro 1x1 rectangular tubing 14 in length:6 ↔ Complete Roller Pneumatic Cylinder Assembly:1
- Mate:639: Vex Pro 1x1 rectangular tubing 14 in length:6 ↔ Complete Roller Pneumatic Cylinder Assembly:1
- Mate:640: Vex Pro 1x1 rectangular tubing 14 in length (roller):1 ↔ Complete Roller Pneumatic Cylinder Assembly:1
- Mate:641: Vex Pro 1x1 rectangular tubing 14 in length (roller):1 ↔ Complete Roller Pneumatic Cylinder Assembly:1
- Mate:642: Vex Pro 1x1 rectangular tubing 14 in length:6 ↔ Vex Pro 90 degree gusset:11
- Mate:644: Vex Pro 1x1 rectangular tubing 14 in length:5 ↔ Complete Roller Pneumatic Cylinder Assembly:2
- Mate:646: Vex Pro 1x1 rectangular tubing 14 in length (roller):2 ↔ Complete Roller Pneumatic Cylinder Assembly:2
- Mate:647: Vex Pro 1x1 rectangular tubing 14 in length (roller):2 ↔ Complete Roller Pneumatic Cylinder Assembly:2
- Mate:648: Vex Pro 1x1 rectangular tubing 14 in length:5 ↔ Complete Roller Pneumatic Cylinder Assembly:2
- Mate:649: Vex Pro 1x1 rectangular tubing 14 in length:5 ↔ Complete Roller Pneumatic Cylinder Assembly:2
## Named parameters: d216_d210 = 0 mm, d217_d213 = 0 mm, d240_d195 = 0 mm, d241_d196 = 0 mm, d242_d197 = 0 mm, d243_d198 = 0 mm, d305_d302 = 0 mm, d306_d303 = 0 mm, d307_d304 = 0 mm, d334_d317 = 0 mm, d335_d318 = -19.05 mm, d336_d325 = 0 mm, d339_d304 = 0 mm, d343_d308 = 0 mm, d344_d309 = 0 mm, d345_d310 = 0 mm, d346_d316 = 0 mm, d347_d326 = 0 mm, d348_d327 = -9.525 mm, d349_d328 = 0 mm, d350_d329 = 0 mm, d351_d330 = 0 mm, d352_d331 = 0 mm, d353_d332 = 0 mm, d354_d333 = 0 mm, d175_d158 = 0 mm, d176_d159 = 0 mm, d177_d160 = 0 mm, d180_d118 = 0 mm, d181_d119 = 0 mm, d182_d120 = 0 mm, d729_d175_d158 = 0 mm, d730_d176_d159 = 0 mm, d731_d177_d160 = 0 mm, d732_d180_d118 = 0 mm, d733_d181_d119 = 0 mm, d734_d182_d120 = 0 mm, d764_d175_d158 = 0 mm, d765_d176_d159 = 0 mm, d766_d177_d160 = 0 mm, d767_d180_d118 = 0 mm, d768_d181_d119 = 0 mm, d769_d182_d120 = 0 mm, d770_d743 = 0 mm, d771_d744 = 0 mm, d772_d745 = 0 mm, d773_d746 = 0 mm, d774_d750 = 2.38125 mm, d781_d729_d175_d158 = 0 mm, d782_d730_d176_d159 = 0 mm, d783_d731_d177_d160 = 0 mm, d784_d732_d180_d118 = 0 mm, d785_d733_d181_d119 = 0 mm, d786_d734_d182_d120 = 0 mm, d787_d738 = 0 mm, d788_d739 = 0 mm, d789_d740 = 0 mm, d790_d741 = 0 mm, d791_d742 = 0 mm
